# Autodesk Inventor assembly: assembledPrototype1
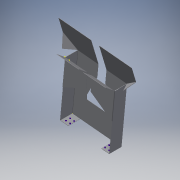
[picture p0: Inventor's stored thumbnail of the model, 180x180]
Saved by Autodesk Inventor 2017 (Build 210142000, 142)
## iProperties
Created: 2017-01-16
Part Number: assembledPrototype1
Document SubType Name: Assembly
Designer: kingb
Author: kingb
## Documents named in this file (4)
- C:\Users\admin\Desktop\CAD\assembledPrototype1.iam
- C:\Users\admin\Desktop\CAD\prototype1(1).ipt
- C:\Users\admin\Desktop\CAD\leftShootGuide.ipt
- C:\Users\admin\Desktop\CAD\rIghtShootGuide.ipt
## Components (3 placed, 3 different names)
1. prototype1(1):1 — Mate:10, Mate:11, Mate:12, Flush:1, Mate:13, Flush:2, Mate:14, Flush:3, Mate:15
2. leftShootGuide:1 — Mate:12, Flush:1, Mate:13
3. rIghtShootGuide:1 — Mate:14, Flush:3, Mate:15
## Relationships (9: Mate 6, Flush 3)
- Mate:10: prototype1(1):1
- Mate:11: prototype1(1):1
- Mate:12: prototype1(1):1 ↔ leftShootGuide:1
- Flush:1: prototype1(1):1 ↔ leftShootGuide:1
- Mate:13: prototype1(1):1 ↔ leftShootGuide:1
- Flush:2 (292.1 mm): prototype1(1):1
- Mate:14: prototype1(1):1 ↔ rIghtShootGuide:1
- Flush:3: prototype1(1):1 ↔ rIghtShootGuide:1
- Mate:15: prototype1(1):1 ↔ rIghtShootGuide:1
